# Autodesk Inventor assembly: Assembly5
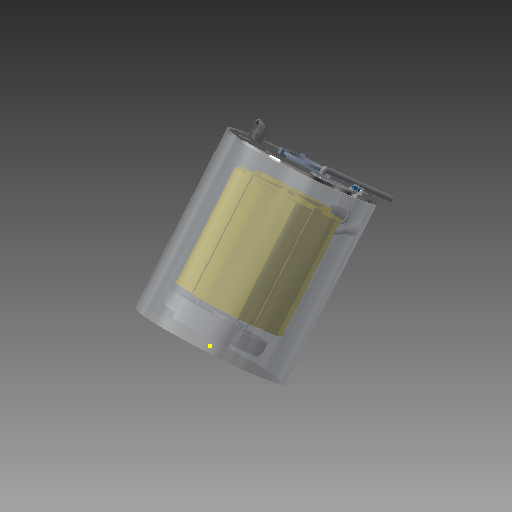
[picture p0: Inventor's stored thumbnail of the model, 512x512]
Saved by Autodesk Inventor 2018 (Build 220112000, 112)
## iProperties
Created: 2021-03-17
Part Number: Assembly5
Document SubType Name: Assembly
Designer: dell
Author: dell
## Documents named in this file (3)
- D:\Autodesk\Projects\C-C\a1\ES101 GROUP-13 PROJECT\FINAL MODEL\Resolved files\Assembly5.iam
- D:\Autodesk\Projects\C-C\a1\ES101 GROUP-13 PROJECT\FINAL MODEL\Resolved files\Assembly4.iam
- D:\Autodesk\Projects\C-C\a1\ES101 GROUP-13 PROJECT\INDIVIDUAL WORK\Tejas\Resolved files\Derived CAP.ipt
## Components (2 placed, 2 different names)
1. Assembly4:1 [sub-assembly] — Mate:1
2. Derived CAP:1 — Mate:1
## Relationships (1: Mate 1)
- Mate:1: Assembly4:1 ↔ Derived CAP:1
